# Autodesk Inventor assembly: Kitchen.02
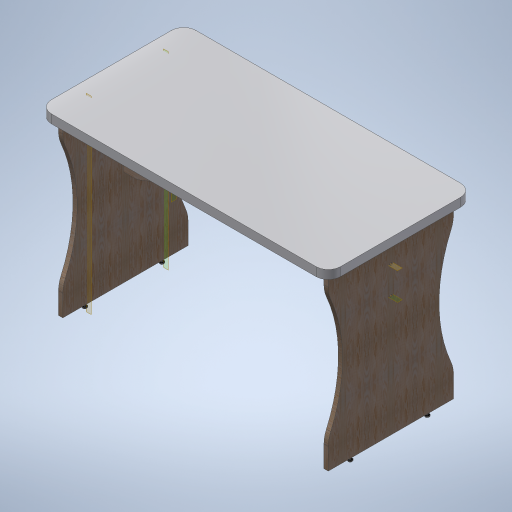
[picture p0: Inventor's stored thumbnail of the model, 512x512]
Saved by Autodesk Inventor 2024 (Build 280153000, 153)
## iProperties
Created: 2016-08-19
Part Number: Kitchen.02
Document SubType Name: Assembly
Designer: SauliusD
Description: Table
Author: SauliusD
## Documents named in this file (12)
- C:\W4INV 2024 Design\PROJECTS\Samples\Simple Kitchen table and stool\Table\Table.iam
- C:\W4INV 2024 Design\PROJECTS\Samples\Simple Kitchen table and stool\Table\Top of Table.ipt
- C:\W4INV 2024 Design\PROJECTS\Samples\Simple Kitchen table and stool\Table\Right Side of Table.ipt
- C:\W4INV 2024 Design\PROJECTS\Samples\Simple Kitchen table and stool\Table\Left Side Of Table.ipt
- C:\W4INV 2024 Design\PROJECTS\Samples\Simple Kitchen table and stool\Table\Confirm of table legs.ipt
- C:\W4INV 2024 Design\_LIBRARY\Fixed joints\Confirmat\CONFIRMAT\Confirmat L50 & Cap D10 NB T18 PB T 18.ipt
- C:\W4INV 2024 Design\_LIBRARY\Fixed joints\Minifix joint\MINIFIX D15 v2\Minifix D15 & Dowel L34 & Cap D15 PB T18 LH.ipt
- C:\W4INV 2024 Design\_LIBRARY\Supports and legs\Supports\ADJUSTABLE SUPPORT\Support M6 H27 D18 with Bushing SB T18.ipt
- C:\W4INV 2024 Design\_LIBRARY\Fixed joints\Minifix joint\MINIFIX D15 v2\Minifix D15 & Dowel L34 & Cap D15 PB T18 RH.ipt
- C:\W4INV 2023 Design\LIBRARY\Fixed joints\Confirmat\CONFIRMAT.ipt
- C:\W4INV 2023 Design\LIBRARY\Fixed joints\Minifix joint\MINIFIX D15 v2.ipt
- C:\W4INV 2023 Design\LIBRARY\Supports and legs\Supports\ADJUSTABLE SUPPORT.ipt
## Components (18 placed, 8 different names)
1. Top of Table:1 — Nestled Board Plane:5, Nestled Board Plane:6, Nestled Board Plane:7, Nestled Board Plane:8, Nestled Board Plane:9, Nestled Board Plane:10
2. Right Side of Table:1 — Nestled Board Plane:1, Nestled Board Plane:3, Pillar Board Side Plane :4, Pillar Board Side Plane :6, Side board:2, Side board:4
3. Left Side Of Table:1 — Flush:5, Flush:6, Nestled Board Plane:2, Nestled Board Plane:4, Pillar Board Side Plane :3, Pillar Board Side Plane :5, Side board:1, Bottom board:1, Bottom board:2, Side board:3, Bottom board:3, Bottom board:4
4. Confirm of table legs:1 — Flush:1, Flush:2, Flush:3, Flush:4, Pillar Board Side Plane:1, Pillar Board Side Plane:2, Pillar Board Side Plane:3, Pillar Board Side Plane:4, Pillar Board Side Plane :1, Pillar Board Side Plane :2
5. Confirmat L50 & Cap D10 NB T18 PB T 18:1 — Axis Plane:1, Nestled Board Plane:1, Pillar Board Side Plane:1
6. Confirmat L50 & Cap D10 NB T18 PB T 18:2 — Axis Plane:2, Nestled Board Plane:2, Pillar Board Side Plane:2
7. Confirmat L50 & Cap D10 NB T18 PB T 18:3 — Axis Plane:3, Nestled Board Plane:3, Pillar Board Side Plane:3
8. Confirmat L50 & Cap D10 NB T18 PB T 18:4 — Axis Plane:4, Nestled Board Plane:4, Pillar Board Side Plane:4
9. Minifix D15 & Dowel L34 & Cap D15 PB T18 LH:1 — Axis Plane:5, Nestled Board Plane:5, Pillar Board Side Plane :1
10. Minifix D15 & Dowel L34 & Cap D15 PB T18 RH:2 — Axis Plane:6, Nestled Board Plane:6, Pillar Board Side Plane :2
11. Minifix D15 & Dowel L34 & Cap D15 PB T18 LH:3 — Axis Plane:7, Pillar Board Side Plane :3, Nestled Board Plane:7
12. Minifix D15 & Dowel L34 & Cap D15 PB T18 RH:4 — Axis Plane:8, Pillar Board Side Plane :4, Nestled Board Plane:8
13. Minifix D15 & Dowel L34 & Cap D15 PB T18 RH:5 — Axis Plane:9, Pillar Board Side Plane :5, Nestled Board Plane:9
14. Minifix D15 & Dowel L34 & Cap D15 PB T18 LH:6 — Axis Plane:10, Pillar Board Side Plane :6, Nestled Board Plane:10
15. Support M6 H27 D18 with Bushing SB T18:1 — Axis:1, Side board:1, Bottom board:1
16. Support M6 H27 D18 with Bushing SB T18:2 — Axis:2, Side board:2, Bottom board:2
17. Support M6 H27 D18 with Bushing SB T18:3 — Axis:3, Side board:3, Bottom board:3
18. Support M6 H27 D18 with Bushing SB T18:4 — Axis:4, Side board:4, Bottom board:4
## Relationships (48: Mate 28, Flush 20)
- Flush:1 (-100 mm): Confirm of table legs:1
- Flush:2 (-100 mm): Confirm of table legs:1
- Flush:3 (-200 mm): Confirm of table legs:1
- Flush:4 (-200 mm): Confirm of table legs:1
- Flush:5 (-100 mm): Left Side Of Table:1
- Flush:6 (-100 mm): Left Side Of Table:1
- Axis Plane:1 [Mate]: Confirmat L50 & Cap D10 NB T18 PB T 18:1
- Nestled Board Plane:1 [Flush]: Right Side of Table:1 ↔ Confirmat L50 & Cap D10 NB T18 PB T 18:1
- Pillar Board Side Plane:1 [Mate] (-9 mm): Confirm of table legs:1 ↔ Confirmat L50 & Cap D10 NB T18 PB T 18:1
- Axis Plane:2 [Mate]: Confirmat L50 & Cap D10 NB T18 PB T 18:2
- Nestled Board Plane:2 [Flush]: Left Side Of Table:1 ↔ Confirmat L50 & Cap D10 NB T18 PB T 18:2
- Pillar Board Side Plane:2 [Mate] (-9 mm): Confirm of table legs:1 ↔ Confirmat L50 & Cap D10 NB T18 PB T 18:2
- Axis Plane:3 [Mate]: Confirmat L50 & Cap D10 NB T18 PB T 18:3
- Nestled Board Plane:3 [Flush]: Right Side of Table:1 ↔ Confirmat L50 & Cap D10 NB T18 PB T 18:3
- Pillar Board Side Plane:3 [Mate] (-9 mm): Confirm of table legs:1 ↔ Confirmat L50 & Cap D10 NB T18 PB T 18:3
- Axis Plane:4 [Mate]: Confirmat L50 & Cap D10 NB T18 PB T 18:4
- Nestled Board Plane:4 [Flush]: Left Side Of Table:1 ↔ Confirmat L50 & Cap D10 NB T18 PB T 18:4
- Pillar Board Side Plane:4 [Mate] (-9 mm): Confirm of table legs:1 ↔ Confirmat L50 & Cap D10 NB T18 PB T 18:4
- Axis Plane:5 [Mate]: Minifix D15 & Dowel L34 & Cap D15 PB T18 LH:1
- Nestled Board Plane:5 [Mate]: Top of Table:1 ↔ Minifix D15 & Dowel L34 & Cap D15 PB T18 LH:1
- Pillar Board Side Plane :1 [Flush] (18 mm): Confirm of table legs:1 ↔ Minifix D15 & Dowel L34 & Cap D15 PB T18 LH:1
- Axis Plane:6 [Mate]: Minifix D15 & Dowel L34 & Cap D15 PB T18 RH:2
- Nestled Board Plane:6 [Mate]: Top of Table:1 ↔ Minifix D15 & Dowel L34 & Cap D15 PB T18 RH:2
- Pillar Board Side Plane :2 [Flush] (18 mm): Confirm of table legs:1 ↔ Minifix D15 & Dowel L34 & Cap D15 PB T18 RH:2
- Axis Plane:7 [Mate]: Minifix D15 & Dowel L34 & Cap D15 PB T18 LH:3
- Pillar Board Side Plane :3 [Flush] (18 mm): Left Side Of Table:1 ↔ Minifix D15 & Dowel L34 & Cap D15 PB T18 LH:3
- Nestled Board Plane:7 [Mate]: Top of Table:1 ↔ Minifix D15 & Dowel L34 & Cap D15 PB T18 LH:3
- Axis Plane:8 [Mate]: Minifix D15 & Dowel L34 & Cap D15 PB T18 RH:4
- Pillar Board Side Plane :4 [Flush] (18 mm): Right Side of Table:1 ↔ Minifix D15 & Dowel L34 & Cap D15 PB T18 RH:4
- Nestled Board Plane:8 [Mate]: Top of Table:1 ↔ Minifix D15 & Dowel L34 & Cap D15 PB T18 RH:4
- Axis Plane:9 [Mate]: Minifix D15 & Dowel L34 & Cap D15 PB T18 RH:5
- Pillar Board Side Plane :5 [Flush] (18 mm): Left Side Of Table:1 ↔ Minifix D15 & Dowel L34 & Cap D15 PB T18 RH:5
- Nestled Board Plane:9 [Mate]: Top of Table:1 ↔ Minifix D15 & Dowel L34 & Cap D15 PB T18 RH:5
- Axis Plane:10 [Mate]: Minifix D15 & Dowel L34 & Cap D15 PB T18 LH:6
- Pillar Board Side Plane :6 [Flush] (18 mm): Right Side of Table:1 ↔ Minifix D15 & Dowel L34 & Cap D15 PB T18 LH:6
- Nestled Board Plane:10 [Mate]: Top of Table:1 ↔ Minifix D15 & Dowel L34 & Cap D15 PB T18 LH:6
- Axis:1 [Mate]: Support M6 H27 D18 with Bushing SB T18:1
- Side board:1 [Flush] (9 mm): Left Side Of Table:1 ↔ Support M6 H27 D18 with Bushing SB T18:1
- Bottom board:1 [Mate] (17.5 mm): Left Side Of Table:1 ↔ Support M6 H27 D18 with Bushing SB T18:1
- Axis:2 [Mate]: Support M6 H27 D18 with Bushing SB T18:2
- Side board:2 [Flush] (9 mm): Right Side of Table:1 ↔ Support M6 H27 D18 with Bushing SB T18:2
- Bottom board:2 [Mate] (17.5 mm): Left Side Of Table:1 ↔ Support M6 H27 D18 with Bushing SB T18:2
- Axis:3 [Mate]: Support M6 H27 D18 with Bushing SB T18:3
- Side board:3 [Flush] (9 mm): Left Side Of Table:1 ↔ Support M6 H27 D18 with Bushing SB T18:3
- Bottom board:3 [Mate] (17.5 mm): Left Side Of Table:1 ↔ Support M6 H27 D18 with Bushing SB T18:3
- Axis:4 [Mate]: Support M6 H27 D18 with Bushing SB T18:4
- Side board:4 [Flush] (9 mm): Right Side of Table:1 ↔ Support M6 H27 D18 with Bushing SB T18:4
- Bottom board:4 [Mate] (17.5 mm): Left Side Of Table:1 ↔ Support M6 H27 D18 with Bushing SB T18:4
